# Autodesk Inventor assembly: E-TEN 1021 On/Off Toggle Switch
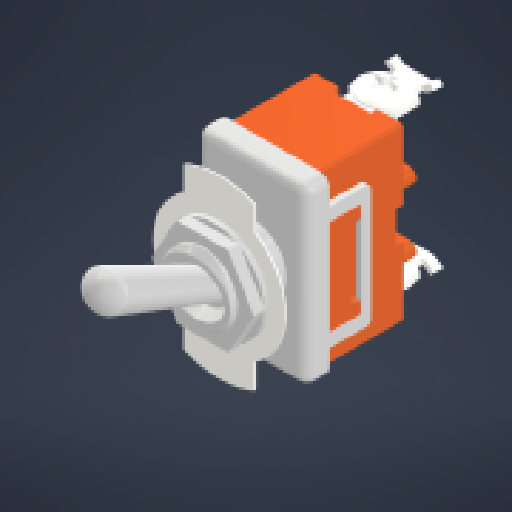
[picture p0: Inventor's stored thumbnail of the model, 512x512]
Saved by Autodesk Inventor 2023 (Build 270158030, 158C)
## iProperties
Created: 2022-04-21
Part Number: E-TEN 1021 On/Off Toggle Switch
Document SubType Name: Assembly
Designer: Norbert Ligas
Sending System: Autodesk Translation Framework v10.14.0.1471
Preprocessor: ST-DEVELOPER v18.1
Title: D:/Documents/_Personal Projects/Electronic Stuff/E-TEN 1021 On-Off Toggle Switch.step
## Documents named in this file (5)
- C:\Users\norbe\Repozytoria\NormalMapScanner\3D_modeling\construction\parts\board_box\Switch\Switch.iam
- C:\Users\norbe\Repozytoria\NormalMapScanner\3D_modeling\construction\parts\board_box\Switch\PanelNut.ipt
- C:\Users\norbe\Repozytoria\NormalMapScanner\3D_modeling\construction\parts\board_box\Switch\On-OffTag.ipt
- C:\Users\norbe\Repozytoria\NormalMapScanner\3D_modeling\construction\parts\board_box\Switch\Washer.ipt
- C:\Users\norbe\Repozytoria\NormalMapScanner\3D_modeling\construction\parts\board_box\Switch\Part9.ipt
## Components (5 placed, 4 different names)
1. Panel Nut:1
2. On-Off Tag:1
3. Washer:1
4. Panel Nut:2
5. Part9
## Named parameters: switch_width = 15.5 mm, switch_length = 29.3 mm, switch_height_with_screws = 28.5 mm, switch_diameter = 12 mm, switch_thread_length = 9 mm
